# Autodesk Inventor assembly: FrameV4
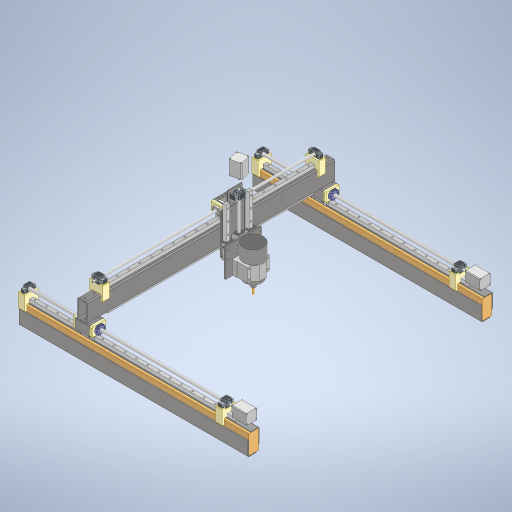
[picture p0: Inventor's stored thumbnail of the model, 512x512]
Saved by Autodesk Inventor 2023 (Build 270158000, 158)
## iProperties
Created: 2022-05-07
Part Number: FrameV4
Document SubType Name: Assembly
Designer: plebbb
Mass: 10930.1 g
Surface Area: 33660.3 cm^2
Volume: 10930.1 cm^3
Density: 1 g/cm^3
Author: plebbb
## Documents named in this file (24)
- C:\Users\think\OneDrive\Desktop\CNC_Project\FrameV4.iam
- C:\Users\think\OneDrive\Desktop\CNC_Project\Ballscrew_Assembly.iam
- C:\Users\think\OneDrive\Desktop\CNC_Project\2x4_Tube.ipt
- C:\Users\think\OneDrive\Desktop\CNC_Project\HGW20CC_Rail_800mm.ipt
- C:\Users\think\OneDrive\Desktop\CNC_Project\BK10.ipt
- C:\Users\think\OneDrive\Desktop\CNC_Project\BF10.ipt
- C:\Users\think\OneDrive\Desktop\CNC_Project\Ballscrew_Assembly_1204.iam
- C:\Users\think\OneDrive\Desktop\CNC_Project\SFU1204-500.ipt
- C:\Users\think\OneDrive\Desktop\CNC_Project\BF10_Spacer.ipt
- C:\Users\think\OneDrive\Desktop\CNC_Project\BK10_Spacer.ipt
- C:\Users\think\OneDrive\Desktop\CNC_Project\2x3_L_Bracket.ipt
- C:\Users\think\OneDrive\Desktop\CNC_Project\HGW20CC_Slider.ipt
- C:\Users\think\OneDrive\Desktop\CNC_Project\Z_Gantry_Plate.ipt
- C:\Users\think\OneDrive\Desktop\CNC_Project\HGW20CC_Rail_300mm.ipt
- C:\Users\think\OneDrive\Desktop\CNC_Project\Rail_Spacer_Plate.ipt
- C:\Users\think\OneDrive\Desktop\CNC_Project\Z_PLATE.iam
- C:\Users\think\OneDrive\Desktop\CNC_Project\SFU1204-300.ipt
- C:\Users\think\OneDrive\Desktop\CNC_Project\Spindle.ipt
- C:\Users\think\OneDrive\Desktop\CNC_Project\Spindle_Holder.ipt
- C:\Users\think\OneDrive\Desktop\CNC_Project\BK10_Z_Mount.ipt
- C:\Users\think\OneDrive\Desktop\CNC_Project\Corner_Brace.ipt
- C:\Users\think\OneDrive\Desktop\CNC_Project\Nema23.ipt
- C:\Users\think\OneDrive\Desktop\CNC_Project\Drill_Bit.ipt
- C:\Users\think\OneDrive\Desktop\CNC_Project\X_GANTRY_WOOD.iam
## Components (30 placed, 23 different names)
1. Ballscrew_Assembly:1 [sub-assembly] — Mate:7, Mate:8, Mate:11, Mate:83
2. Ballscrew_Assembly:2 [sub-assembly] — Mate:9, Mate:10, Mate:12, Mate:81, Mate:82
3. 2x4_Tube:1 — Mate:7, Mate:8, Mate:9, Mate:10, Mate:11, Mate:12, Flush:4, Mate:15, Mate:26, Mate:27, Mate:34, Mate:35, Flush:5, Mate:45
4. HGW20CC_Rail_800mm:1 — Flush:4, Mate:15, Mate:22, Mate:23, Mate:38, Flush:6, Flush:7
5. BK10:1 — Mate:40, Mate:41, Mate:42, Mate:43, Mate:44
6. BF10:1 — Mate:31, Mate:32, Mate:33, Mate:36
7. Ballscrew_Assembly_1204:1 [sub-assembly] — Mate:22, Mate:23, Mate:24, Mate:39, Mate:44, Mate:51, Mate:52, Mate:54, Mate:68, Angle:3
8. SFU1204-500:1 — Mate:24, Mate:36, Mate:43
9. BF10_Spacer:1 — Mate:31, Mate:32, Mate:33, Mate:34, Mate:35, Flush:5, Mate:38, Mate:39
10. BK10_Spacer:1 — Mate:26, Mate:27, Mate:40, Mate:41, Mate:42
11. HGW20CC_Rail_800mm:2 — Flush:6, Mate:45, Mate:49, Mate:50, Flush:7
12. 2x3_L_Bracket:1 — Mate:46, Mate:47, Mate:48, Mate:53
13. HGW20CC_Slider:1 — Mate:46, Mate:47, Mate:48, Mate:49, Mate:50
14. Z_Gantry_Plate:1 — Mate:51, Mate:52, Mate:53, Mate:54, Angle:2, Mate:55, Mate:56, Flush:9, Flush:10, Flush:12, Flush:14, Flush:15, Flush:17
15. HGW20CC_Rail_300mm:1 — Flush:8, Angle:1, Angle:2, Mate:57, Flush:11, Flush:12, Flush:16
16. HGW20CC_Rail_300mm:2 — Flush:8, Angle:1, Mate:58, Flush:13, Flush:14, Flush:15, Mate:59, Mate:60
17. Rail_Spacer_Plate:1 — Mate:55, Flush:9, Mate:57, Flush:11
18. Rail_Spacer_Plate:2 — Mate:56, Flush:10, Mate:58, Flush:13
19. Z_PLATE:1 [sub-assembly] — Mate:59, Mate:60, Flush:16, Mate:61, Mate:63, Mate:64, Mate:65, Mate:77
20. SFU1204-300:1 — Mate:61, Flush:17, Mate:66, Mate:67, Mate:74
21. Spindle:1 — Mate:62, Flush:18, Mate:75, Mate:76
22. Spindle_Holder:1 — Mate:62, Flush:18, Mate:63, Mate:64, Mate:65
23. BK10:2 — Mate:66, Mate:67, Mate:69, Mate:77, Mate:78, Mate:79
24. BK10_Z_Mount:1 — Mate:68, Mate:69, Angle:3, Mate:70, Mate:71, Mate:72, Mate:73, Flush:19, Flush:20, Mate:78, Mate:79
25. Corner_Brace:1 — Mate:71, Mate:72, Flush:19
26. Corner_Brace:2 — Mate:70, Mate:73, Flush:20
27. Nema23:1 — Mate:74
28. Drill_Bit:1 — Mate:75, Mate:76
29. X_GANTRY_WOOD:1 [sub-assembly] — Mate:81, Mate:82, Flush:82, Flush:83
30. X_GANTRY_WOOD:2 [sub-assembly] — Flush:81, Flush:21, Mate:80, Mate:83, Flush:82, Flush:83
## Relationships (88: Mate 64, Flush 21, Angle 3)
- Mate:7: Ballscrew_Assembly:1 ↔ 2x4_Tube:1
- Mate:8: Ballscrew_Assembly:1 ↔ 2x4_Tube:1
- Mate:9: Ballscrew_Assembly:2 ↔ 2x4_Tube:1
- Mate:10: Ballscrew_Assembly:2 ↔ 2x4_Tube:1
- Mate:11: Ballscrew_Assembly:1 ↔ 2x4_Tube:1
- Mate:12: Ballscrew_Assembly:2 ↔ 2x4_Tube:1
- Flush:4 (15.4 mm): 2x4_Tube:1 ↔ HGW20CC_Rail_800mm:1
- Mate:15: 2x4_Tube:1 ↔ HGW20CC_Rail_800mm:1
- Mate:22: HGW20CC_Rail_800mm:1 ↔ Ballscrew_Assembly_1204:1
- Mate:23: HGW20CC_Rail_800mm:1 ↔ Ballscrew_Assembly_1204:1
- Mate:24: Ballscrew_Assembly_1204:1 ↔ SFU1204-500:1
- Mate:26: 2x4_Tube:1 ↔ BK10_Spacer:1
- Mate:27: 2x4_Tube:1 ↔ BK10_Spacer:1
- Mate:31: BF10:1 ↔ BF10_Spacer:1
- Mate:32: BF10:1 ↔ BF10_Spacer:1
- Mate:33: BF10:1 ↔ BF10_Spacer:1
- Mate:34: 2x4_Tube:1 ↔ BF10_Spacer:1
- Mate:35: 2x4_Tube:1 ↔ BF10_Spacer:1
- Mate:36: BF10:1 ↔ SFU1204-500:1
- Flush:5 (60 mm): 2x4_Tube:1 ↔ BF10_Spacer:1
- Mate:38: HGW20CC_Rail_800mm:1 ↔ BF10_Spacer:1
- Mate:39: Ballscrew_Assembly_1204:1 ↔ BF10_Spacer:1
- Mate:40: BK10:1 ↔ BK10_Spacer:1
- Mate:41: BK10:1 ↔ BK10_Spacer:1
- Mate:42: BK10:1 ↔ BK10_Spacer:1
- Mate:43: BK10:1 ↔ SFU1204-500:1
- Mate:44: BK10:1 ↔ Ballscrew_Assembly_1204:1
- Flush:6: HGW20CC_Rail_800mm:1 ↔ HGW20CC_Rail_800mm:2
- Mate:45: 2x4_Tube:1 ↔ HGW20CC_Rail_800mm:2
- Mate:46: 2x3_L_Bracket:1 ↔ HGW20CC_Slider:1
- Mate:47: 2x3_L_Bracket:1 ↔ HGW20CC_Slider:1
- Mate:48: 2x3_L_Bracket:1 ↔ HGW20CC_Slider:1
- Mate:49: HGW20CC_Rail_800mm:2 ↔ HGW20CC_Slider:1
- Mate:50: HGW20CC_Rail_800mm:2 ↔ HGW20CC_Slider:1
- Flush:7: HGW20CC_Rail_800mm:1 ↔ HGW20CC_Rail_800mm:2
- Mate:51: Ballscrew_Assembly_1204:1 ↔ Z_Gantry_Plate:1
- Mate:52: Ballscrew_Assembly_1204:1 ↔ Z_Gantry_Plate:1
- Mate:53: 2x3_L_Bracket:1 ↔ Z_Gantry_Plate:1
- Mate:54: Ballscrew_Assembly_1204:1 ↔ Z_Gantry_Plate:1
- Flush:8: HGW20CC_Rail_300mm:1 ↔ HGW20CC_Rail_300mm:2
- Angle:1 (0 deg): HGW20CC_Rail_300mm:1 ↔ HGW20CC_Rail_300mm:2
- Angle:2 (0 deg): Z_Gantry_Plate:1 ↔ HGW20CC_Rail_300mm:1
- Mate:55: Z_Gantry_Plate:1 ↔ Rail_Spacer_Plate:1
- Mate:56: Z_Gantry_Plate:1 ↔ Rail_Spacer_Plate:2
- Flush:9: Z_Gantry_Plate:1 ↔ Rail_Spacer_Plate:1
- Flush:10: Z_Gantry_Plate:1 ↔ Rail_Spacer_Plate:2
- Mate:57: HGW20CC_Rail_300mm:1 ↔ Rail_Spacer_Plate:1
- Mate:58: HGW20CC_Rail_300mm:2 ↔ Rail_Spacer_Plate:2
- Flush:11: HGW20CC_Rail_300mm:1 ↔ Rail_Spacer_Plate:1
- Flush:12 (5.2 mm): Z_Gantry_Plate:1 ↔ HGW20CC_Rail_300mm:1
- Flush:13: HGW20CC_Rail_300mm:2 ↔ Rail_Spacer_Plate:2
- Flush:14 (5.2 mm): Z_Gantry_Plate:1 ↔ HGW20CC_Rail_300mm:2
- Flush:15: Z_Gantry_Plate:1 ↔ HGW20CC_Rail_300mm:2
- Mate:59: HGW20CC_Rail_300mm:2 ↔ Z_PLATE:1
- Mate:60: HGW20CC_Rail_300mm:2 ↔ Z_PLATE:1
- Flush:16: HGW20CC_Rail_300mm:1 ↔ Z_PLATE:1
- Mate:61: Z_PLATE:1 ↔ SFU1204-300:1
- Flush:17: Z_Gantry_Plate:1 ↔ SFU1204-300:1
- Mate:62: Spindle:1 ↔ Spindle_Holder:1
- Flush:18 (-20 mm): Spindle:1 ↔ Spindle_Holder:1
- Mate:63: Z_PLATE:1 ↔ Spindle_Holder:1
- Mate:64: Z_PLATE:1 ↔ Spindle_Holder:1
- Mate:65: Z_PLATE:1 ↔ Spindle_Holder:1
- Mate:66: SFU1204-300:1 ↔ BK10:2
- Mate:67: SFU1204-300:1 ↔ BK10:2
- Mate:68: Ballscrew_Assembly_1204:1 ↔ BK10_Z_Mount:1
- Mate:69: BK10:2 ↔ BK10_Z_Mount:1
- Angle:3 (180 deg): Ballscrew_Assembly_1204:1 ↔ BK10_Z_Mount:1
- Mate:70: BK10_Z_Mount:1 ↔ Corner_Brace:2
- Mate:71: BK10_Z_Mount:1 ↔ Corner_Brace:1
- Mate:72: BK10_Z_Mount:1 ↔ Corner_Brace:1
- Mate:73: BK10_Z_Mount:1 ↔ Corner_Brace:2
- Flush:19: BK10_Z_Mount:1 ↔ Corner_Brace:1
- Flush:20: BK10_Z_Mount:1 ↔ Corner_Brace:2
- Mate:74: SFU1204-300:1 ↔ Nema23:1
- Mate:75: Spindle:1 ↔ Drill_Bit:1
- Mate:76: Spindle:1 ↔ Drill_Bit:1
- Mate:77 (10 mm): Z_PLATE:1 ↔ BK10:2
- Mate:78: BK10:2 ↔ BK10_Z_Mount:1
- Mate:79: BK10:2 ↔ BK10_Z_Mount:1
- Flush:81: X_GANTRY_WOOD:2
- Flush:21: X_GANTRY_WOOD:2
- Mate:80: X_GANTRY_WOOD:2
- Mate:81: Ballscrew_Assembly:2 ↔ X_GANTRY_WOOD:1
- Mate:82: Ballscrew_Assembly:2 ↔ X_GANTRY_WOOD:1
- Mate:83: Ballscrew_Assembly:1 ↔ X_GANTRY_WOOD:2
- Flush:82: X_GANTRY_WOOD:1 ↔ X_GANTRY_WOOD:2
- Flush:83: X_GANTRY_WOOD:1 ↔ X_GANTRY_WOOD:2
